# Autodesk Inventor assembly: Pi Cam and Cable assembly
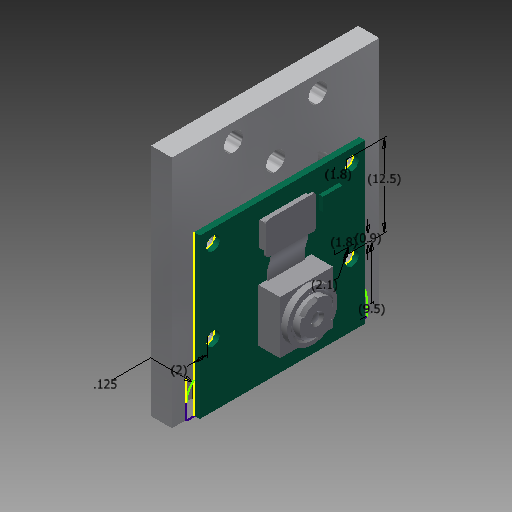
[picture p0: Inventor's stored thumbnail of the model, 512x512]
Saved by Autodesk Inventor 2017 (Build 210142000, 142)
## iProperties
Created: 2017-01-19
Part Number: Pi Cam and Cable assembly
Document SubType Name: Assembly
Designer: qupec
Author: qupec
## Documents named in this file (4)
- C:\UMD\BPP\ROCKSAT X\star\CAD\Mechanical\Full payload assembly\Subsystems\Video Capture\Pi Cam and Cable assembly.iam
- C:\UMD\BPP\ROCKSAT X\star\CAD\Mechanical\Full payload assembly\Subsystems\Pi Cam\Raspberry Pi Camera.iam
- C:\UMD\BPP\ROCKSAT X\star\CAD\Mechanical\Full payload assembly\Subsystems\Electronics\Ribbon Cable Connector-01.ipt
- C:\UMD\BPP\ROCKSAT X\star\CAD\Mechanical\Full payload assembly\Subsystems\Video Capture\Camera Mount.ipt
## Components (3 placed, 3 different names)
1. Raspberry Pi Camera:1 [sub-assembly] — Mate:1, Flush:1, Flush:2, Mate:2, Mate:3, Mate:4
2. Ribbon Cable Connector-01:2 — Mate:1, Flush:1, Flush:2
3. Camera Mount:1 — Mate:2, Mate:3, Mate:4
## Relationships (6: Mate 4, Flush 2)
- Mate:1: Raspberry Pi Camera:1 ↔ Ribbon Cable Connector-01:2
- Flush:1 (2.1 mm): Raspberry Pi Camera:1 ↔ Ribbon Cable Connector-01:2
- Flush:2: Raspberry Pi Camera:1 ↔ Ribbon Cable Connector-01:2
- Mate:2: Raspberry Pi Camera:1 ↔ Camera Mount:1
- Mate:3: Raspberry Pi Camera:1 ↔ Camera Mount:1
- Mate:4: Raspberry Pi Camera:1 ↔ Camera Mount:1
